# Autodesk Inventor assembly: frame_test_assembly
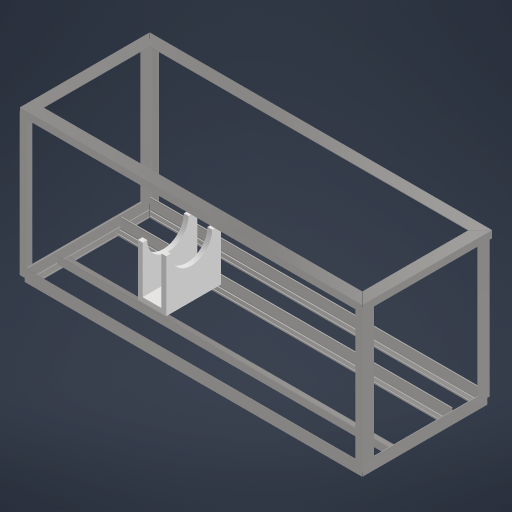
[picture p0: Inventor's stored thumbnail of the model, 512x512]
Saved by Autodesk Inventor 2023 (Build 270158000, 158)
## iProperties
_SolveAssemblyDoc: Frame Generator Solve Assembly
_Version: 25.0.0
Created: 2022-09-07
Part Number: frame_test_assembly
Document SubType Name: Assembly
Designer: Mike
Author: Mike
## Documents named in this file (4)
- C:\Users\Mike\Desktop\Mechatronics\Mechatronics 5.1\Liquid-engine-cooling-system\design files\Ethanol engine 5 -inventor files\frame_test_assembly.iam
- C:\Users\Mike\Desktop\Mechatronics\Mechatronics 5.1\Liquid-engine-cooling-system\design files\Ethanol engine 5 -inventor files\testhell.ipt
- C:\Users\Mike\Desktop\Mechatronics\Mechatronics 5.1\Liquid-engine-cooling-system\design files\Ethanol engine 5 -inventor files\frame_test_assembly\Frame\Frame 1662558230111.iam
- C:\Users\Mike\Desktop\Mechatronics\Mechatronics 5.1\Liquid-engine-cooling-system\design files\Ethanol engine 5 -inventor files\support assembly.iam
## Components (3 placed, 3 different names)
1. testhell:1 — Mate:1, Mate:2
2. Frame 1662558230111:1 [sub-assembly]
3. support assembly:1 [sub-assembly] — Mate:1, Mate:2
## Relationships (2: Mate 2)
- Mate:1: testhell:1 ↔ support assembly:1
- Mate:2: testhell:1 ↔ support assembly:1
